# Autodesk Inventor assembly: final assembly
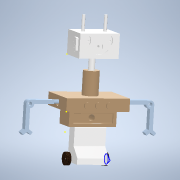
[picture p0: Inventor's stored thumbnail of the model, 180x180]
Saved by Autodesk Inventor 2021 (Build 250183000, 183)
## iProperties
Created: 2021-07-11
Part Number: final assembly
Document SubType Name: Assembly
Designer: 91968
Author: 91968
## Documents named in this file (6)
- E:\BME\INVENTOR_FILES\interactive toy\final assembly.iam
- E:\BME\INVENTOR_FILES\interactive toy\body (2).ipt
- C:\Users\91968\Downloads\leg (2).ipt
- C:\Users\91968\Downloads\head part 2.ipt
- C:\Users\91968\Downloads\wheel (1).ipt
- C:\Users\91968\Downloads\Hand 4.ipt
## Components (7 placed, 5 different names)
1. body (2):1 — Rigid:2, Rigid:3, Rigid:4, Rigid:5
2. leg (2):1 — Rigid:2, Rotational:1, Rotational:2
3. wheel (1):1 — Rotational:2
4. Hand 4:1 — Rigid:4
5. Hand 4:2 — Rigid:5
6. head part 2:2 — Rigid:3
7. wheel (1):3 — Rotational:1
## Relationships (6: WeldJoint 4, RevoluteJoint 2)
- Rigid:2 [WeldJoint]: body (2):1 ↔ leg (2):1
- Rigid:3 [WeldJoint]: body (2):1 ↔ head part 2:2
- Rigid:4 [WeldJoint]: body (2):1 ↔ Hand 4:1
- Rigid:5 [WeldJoint]: body (2):1 ↔ Hand 4:2
- Rotational:1 [RevoluteJoint]: leg (2):1 ↔ wheel (1):3
- Rotational:2 [RevoluteJoint]: leg (2):1 ↔ wheel (1):1
